# Autodesk Inventor assembly: 总1
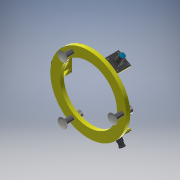
[picture p0: Inventor's stored thumbnail of the model, 180x180]
Saved by Autodesk Inventor 2017 (Build 210142000, 142)
## iProperties
Part Number: 总1
Material: 常规
Document SubType Name: Assembly
Designer: Administrator
Author: Administrator
## Documents named in this file (8)
- D:\大四上\传感器\小轿车\总1.iam
- D:\大四上\传感器\小轿车\镜头.ipt
- D:\大四上\传感器\小轿车\相机.ipt
- D:\大四上\传感器\小轿车\支座.ipt
- C:\Users\Administrator\Documents\Inventor\Content Center Files\R2017\zh-CN\GB_T 70.1\螺钉 GB_T 70.1 M1.6 x 8.ipt
- C:\Users\Administrator\Documents\Inventor\Content Center Files\R2017\zh-CN\GB_T 6170-2000\螺母 GB_T 6170 M1.6.ipt
- C:\Users\Administrator\Documents\Inventor\Content Center Files\R2017\zh-CN\GB_T 70.1\螺钉 GB_T 70.1 M12 x 30.ipt
- D:\大四上\传感器\小轿车\吸盘.ipt
## Components (37 placed, 7 different names)
1. 镜头:1 — 配合:1, 配合:2
2. 相机:1 — 配合:1, 配合:2, 配合:13, 配合:14, 配合:15
3. 镜头:2
4. 相机:2 — 配合:10, 配合:11, 配合:12, 插入:1, 插入:2, 插入:3, 插入:4
5. 镜头:3
6. 相机:3 — 配合:7, 配合:8, 配合:9
7. 支座:1 — 配合:7, 配合:8, 配合:9, 配合:10, 配合:11, 配合:12, 配合:13, 配合:14, 配合:15, 插入:5, 插入:6, 插入:7, 插入:8, 插入:9, 插入:10, 插入:11
8. 螺钉 GB/T 70.1 M12 x 30:1 — 插入:9, 配合:16, 配合:17
9. 螺钉 GB/T 70.1 M12 x 30:2 — 插入:10
10. 螺钉 GB/T 70.1 M12 x 30:3 — 插入:11
11. 螺钉 GB/T 70.1 M1.6 x 8:1 — 插入:1
12. 螺钉 GB/T 70.1 M1.6 x 8:2 — 插入:2
13. 螺钉 GB/T 70.1 M1.6 x 8:3 — 插入:3
14. 螺钉 GB/T 70.1 M1.6 x 8:4 — 插入:4
15. 螺母 GB/T 6170-2000 M1.6:1 — 插入:5
16. 螺母 GB/T 6170-2000 M1.6:2 — 插入:6
17. 螺母 GB/T 6170-2000 M1.6:3 — 插入:7
18. 螺母 GB/T 6170-2000 M1.6:4 — 插入:8
19. 螺钉 GB/T 70.1 M1.6 x 8:5
20. 螺钉 GB/T 70.1 M1.6 x 8:6
21. 螺钉 GB/T 70.1 M1.6 x 8:7
22. 螺钉 GB/T 70.1 M1.6 x 8:8
23. 螺母 GB/T 6170-2000 M1.6:5
24. 螺母 GB/T 6170-2000 M1.6:6
25. 螺母 GB/T 6170-2000 M1.6:7
26. 螺母 GB/T 6170-2000 M1.6:8
27. 螺钉 GB/T 70.1 M1.6 x 8:9
28. 螺钉 GB/T 70.1 M1.6 x 8:10
29. 螺钉 GB/T 70.1 M1.6 x 8:11
30. 螺钉 GB/T 70.1 M1.6 x 8:12
31. 螺母 GB/T 6170-2000 M1.6:9
32. 螺母 GB/T 6170-2000 M1.6:10
33. 螺母 GB/T 6170-2000 M1.6:11
34. 螺母 GB/T 6170-2000 M1.6:12
35. 吸盘:2 — 配合:16, 配合:17
36. 吸盘:3
37. 吸盘:4
## Component patterns: (3 elements, first: 螺钉 GB/T 70.1 M1.6 x 8:1 + 螺钉 GB/T 70.1 M1.6 x 8:2 + 螺钉 GB/T 70.1 M1.6 x 8:3 + 螺钉 GB/T 70.1 M1.6 x 8:4 + 螺母 GB/T 6170-2000 M1.6:1 + 螺母 GB/T 6170-2000 M1.6:2 + 螺母 GB/T 6170-2000 M1.6:3 + 螺母 GB/T 6170-2000 M1.6:4), (3 elements, first: 吸盘:2)
## Relationships (28: Mate 17, Insert 11)
- 配合:1 [Mate]: 镜头:1 ↔ 相机:1
- 配合:2 [Mate]: 镜头:1 ↔ 相机:1
- [Mate]: 镜头:2 ↔ 相机:2
- [Mate]: 镜头:2 ↔ 相机:2
- [Mate]: 镜头:3 ↔ 相机:3
- [Mate]: 镜头:3 ↔ 相机:3
- 配合:7 [Mate]: 相机:3 ↔ 支座:1
- 配合:8 [Mate]: 相机:3 ↔ 支座:1
- 配合:9 [Mate]: 相机:3 ↔ 支座:1
- 配合:10 [Mate]: 相机:2 ↔ 支座:1
- 配合:11 [Mate]: 相机:2 ↔ 支座:1
- 配合:12 [Mate]: 相机:2 ↔ 支座:1
- 配合:13 [Mate]: 相机:1 ↔ 支座:1
- 配合:14 [Mate]: 相机:1 ↔ 支座:1
- 配合:15 [Mate]: 相机:1 ↔ 支座:1
- 插入:1 [Insert]: 相机:2 ↔ 螺钉 GB/T 70.1 M1.6 x 8:1
- 插入:2 [Insert]: 相机:2 ↔ 螺钉 GB/T 70.1 M1.6 x 8:2
- 插入:3 [Insert]: 相机:2 ↔ 螺钉 GB/T 70.1 M1.6 x 8:3
- 插入:4 [Insert]: 相机:2 ↔ 螺钉 GB/T 70.1 M1.6 x 8:4
- 插入:5 [Insert]: 支座:1 ↔ 螺母 GB/T 6170-2000 M1.6:1
- 插入:6 [Insert]: 支座:1 ↔ 螺母 GB/T 6170-2000 M1.6:2
- 插入:7 [Insert]: 支座:1 ↔ 螺母 GB/T 6170-2000 M1.6:3
- 插入:8 [Insert]: 支座:1 ↔ 螺母 GB/T 6170-2000 M1.6:4
- 插入:9 [Insert]: 支座:1 ↔ 螺钉 GB/T 70.1 M12 x 30:1
- 插入:10 [Insert]: 支座:1 ↔ 螺钉 GB/T 70.1 M12 x 30:2
- 插入:11 [Insert]: 支座:1 ↔ 螺钉 GB/T 70.1 M12 x 30:3
- 配合:16 [Mate]: 螺钉 GB/T 70.1 M12 x 30:1 ↔ 吸盘:2
- 配合:17 [Mate]: 螺钉 GB/T 70.1 M12 x 30:1 ↔ 吸盘:2
## Named parameters: d2_d0 = 0 mm, d3_d1 = 0 mm, d4_d0 = 0 mm, d5_d1 = 0 mm
